# Autodesk Inventor assembly: B_Foot_v2
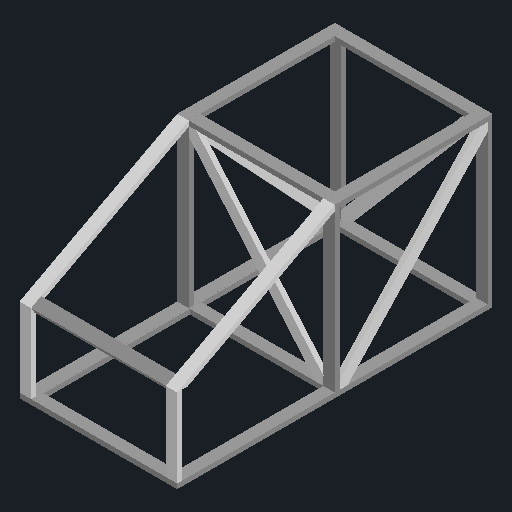
[picture p0: Inventor's stored thumbnail of the model, 512x512]
Saved by Autodesk Inventor 2027.1 (Build 311270010, 270A)
## iProperties
Created: 2026-08-30
Part Number: B_Foot_v2
Document SubType Name: Assembly
Designer: jorda
Author: jorda
## Documents named in this file (8)
- C:\Users\jorda\OneDrive\Documents\GitHub\USC-ASME-TigerBurn-2026\CAD\Legs\Back Foot\B_Foot_v2.iam
- C:\Users\jorda\OneDrive\Documents\GitHub\USC-ASME-TigerBurn-2026\CAD\Legs\Back Foot\2x4x96.ipt
- C:\Users\jorda\OneDrive\Documents\GitHub\USC-ASME-TigerBurn-2026\CAD\Legs\Back Foot\2x4x42.ipt
- C:\Users\jorda\OneDrive\Documents\GitHub\USC-ASME-TigerBurn-2026\CAD\Legs\Back Foot\2x4x48.ipt
- C:\Users\jorda\OneDrive\Documents\GitHub\USC-ASME-TigerBurn-2026\CAD\Legs\Back Foot\2x4x30.ipt
- C:\Users\jorda\OneDrive\Documents\GitHub\USC-ASME-TigerBurn-2026\CAD\Legs\Back Foot\S_2x4x54.35.ipt
- C:\Users\jorda\OneDrive\Documents\GitHub\USC-ASME-TigerBurn-2026\CAD\Legs\Back Foot\S_2x4x65.8.ipt
- C:\Users\jorda\OneDrive\Documents\GitHub\USC-ASME-TigerBurn-2026\CAD\Legs\Back Foot\S_2x4x63.13.ipt
## Components (24 placed, 7 different names)
1. 2x4x96:2 — Mate:1, Flush:1, Flush:2, Flush:3, Mate:2, Flush:4, Mate:4, Flush:7, Flush:8, Flush:24, Flush:27, Flush:28
2. 2x4x42:1 — Mate:1, Flush:1, Flush:2, Flush:10
3. 2x4x42:2 — Flush:3, Mate:2, Flush:4, Flush:5, Flush:6, Mate:3, Flush:25, Mate:12, Mate:13
4. 2x4x96:3 — Flush:5, Flush:6, Mate:3, Flush:9, Mate:5, Flush:26, Mate:19, Flush:32
5. 2x4x48:1 — Mate:4, Flush:7, Flush:8, Mate:7, Flush:13, Flush:14
6. 2x4x48:2 — Flush:9, Flush:10, Mate:5, Flush:11, Flush:12, Mate:6, Mate:22, Flush:34, Mate:26
7. 2x4x48:3 — Flush:11, Flush:12, Mate:6, Flush:15, Flush:16, Flush:17, Mate:10, Mate:14
8. 2x4x48:4 — Mate:7, Flush:13, Flush:14, Flush:18, Flush:19, Mate:8, Flush:20, Flush:21, Mate:9, Flush:23, Mate:15, Flush:30, Mate:21, Flush:33
9. 2x4x48:5 — Flush:15, Flush:16, Flush:17, Flush:29, Mate:18
10. 2x4x48:6 — Flush:18, Flush:19, Mate:8, Flush:22, Mate:11, Mate:20, Mate:24, Flush:35
11. 2x4x42:3 — Flush:20, Flush:21, Mate:9, Mate:23
12. 2x4x42:4 — Flush:22, Flush:23, Mate:10, Mate:25
13. 2x4x42:5 — Mate:11, Flush:24
14. 2x4x30:1 — Flush:25, Flush:26, Mate:12, Flush:36
15. 2x4x30:2 — Flush:27, Flush:28, Mate:13, Mate:27, Flush:37
16. S_2x4x54.35:1 — Mate:14, Flush:29, Mate:16, Mate:17
17. S_2x4x54.35:2 — Mate:15, Flush:30, Flush:31
18. 2x4x42:6 — Flush:31, Mate:16, Mate:17
19. S_2x4x65.8:1 — Mate:18, Mate:19, Flush:32
20. S_2x4x65.8:2 — Mate:20, Mate:21, Flush:33
21. S_2x4x63.13:1 — Mate:22, Mate:23, Flush:34
22. S_2x4x63.13:2 — Mate:24, Flush:35, Mate:25
23. 2x4x96:1 — Mate:26, Flush:36
24. 2x4x96:2 — Mate:27, Flush:37
## Relationships (64: Flush 37, Mate 27)
- Mate:1: 2x4x96:2 ↔ 2x4x42:1
- Flush:1: 2x4x96:2 ↔ 2x4x42:1
- Flush:2: 2x4x96:2 ↔ 2x4x42:1
- Flush:3: 2x4x96:2 ↔ 2x4x42:2
- Mate:2: 2x4x96:2 ↔ 2x4x42:2
- Flush:4: 2x4x96:2 ↔ 2x4x42:2
- Flush:5: 2x4x42:2 ↔ 2x4x96:3
- Flush:6: 2x4x42:2 ↔ 2x4x96:3
- Mate:3: 2x4x42:2 ↔ 2x4x96:3
- Mate:4: 2x4x96:2 ↔ 2x4x48:1
- Flush:7: 2x4x96:2 ↔ 2x4x48:1
- Flush:8: 2x4x96:2 ↔ 2x4x48:1
- Flush:9: 2x4x96:3 ↔ 2x4x48:2
- Flush:10: 2x4x42:1 ↔ 2x4x48:2
- Mate:5: 2x4x96:3 ↔ 2x4x48:2
- Flush:11: 2x4x48:2 ↔ 2x4x48:3
- Flush:12: 2x4x48:2 ↔ 2x4x48:3
- Mate:6: 2x4x48:2 ↔ 2x4x48:3
- Mate:7: 2x4x48:1 ↔ 2x4x48:4
- Flush:13: 2x4x48:1 ↔ 2x4x48:4
- Flush:14: 2x4x48:1 ↔ 2x4x48:4
- Flush:15: 2x4x48:3 ↔ 2x4x48:5
- Flush:16: 2x4x48:3 ↔ 2x4x48:5
- Flush:17: 2x4x48:3 ↔ 2x4x48:5
- Flush:18: 2x4x48:4 ↔ 2x4x48:6
- Flush:19: 2x4x48:4 ↔ 2x4x48:6
- Mate:8: 2x4x48:4 ↔ 2x4x48:6
- Flush:20: 2x4x48:4 ↔ 2x4x42:3
- Flush:21: 2x4x48:4 ↔ 2x4x42:3
- Mate:9: 2x4x48:4 ↔ 2x4x42:3
- Flush:22: 2x4x48:6 ↔ 2x4x42:4
- Flush:23: 2x4x48:4 ↔ 2x4x42:4
- Mate:10: 2x4x48:3 ↔ 2x4x42:4
- Mate:11: 2x4x48:6 ↔ 2x4x42:5
- Flush:24: 2x4x96:2 ↔ 2x4x42:5
- Flush:25: 2x4x42:2 ↔ 2x4x30:1
- Flush:26: 2x4x96:3 ↔ 2x4x30:1
- Mate:12: 2x4x42:2 ↔ 2x4x30:1
- Flush:27: 2x4x96:2 ↔ 2x4x30:2
- Flush:28: 2x4x96:2 ↔ 2x4x30:2
- Mate:13: 2x4x42:2 ↔ 2x4x30:2
- Mate:14: 2x4x48:3 ↔ S_2x4x54.35:1
- Flush:29: 2x4x48:5 ↔ S_2x4x54.35:1
- Mate:15: 2x4x48:4 ↔ S_2x4x54.35:2
- Flush:30: 2x4x48:4 ↔ S_2x4x54.35:2
- Flush:31: S_2x4x54.35:2 ↔ 2x4x42:6
- Mate:16: S_2x4x54.35:1 ↔ 2x4x42:6
- Mate:17: S_2x4x54.35:1 ↔ 2x4x42:6
- Mate:18: 2x4x48:5 ↔ S_2x4x65.8:1
- Mate:19: 2x4x96:3 ↔ S_2x4x65.8:1
- Flush:32: 2x4x96:3 ↔ S_2x4x65.8:1
- Mate:20: 2x4x48:6 ↔ S_2x4x65.8:2
- Mate:21: 2x4x48:4 ↔ S_2x4x65.8:2
- Flush:33: 2x4x48:4 ↔ S_2x4x65.8:2
- Mate:22: 2x4x48:2 ↔ S_2x4x63.13:1
- Mate:23: 2x4x42:3 ↔ S_2x4x63.13:1
- Flush:34: 2x4x48:2 ↔ S_2x4x63.13:1
- Mate:24: 2x4x48:6 ↔ S_2x4x63.13:2
- Flush:35: 2x4x48:6 ↔ S_2x4x63.13:2
- Mate:25: 2x4x42:4 ↔ S_2x4x63.13:2
- Mate:26: 2x4x48:2 ↔ 2x4x96:1
- Flush:36: 2x4x30:1 ↔ 2x4x96:1
- Mate:27: 2x4x30:2 ↔ 2x4x96:2
- Flush:37: 2x4x30:2 ↔ 2x4x96:2
